# Autodesk Inventor assembly: left arm
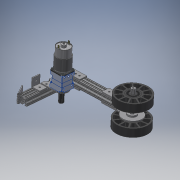
[picture p0: Inventor's stored thumbnail of the model, 180x180]
Saved by Autodesk Inventor 2018 (Build 220112000, 112)
## iProperties
Created: 2019-01-25
Part Number: left arm
Document SubType Name: Assembly
Designer: s-2513225
Author: s-2513225
## Documents named in this file (12)
- E:\Robotics\Ball Intake ver 2\left arm.iam
- E:\Robotics\Ball Intake ver 2\1010 6in.ipt
- E:\Robotics\Ball Intake ver 2\1010 7in.ipt
- E:\Robotics\Ball Intake ver 2\motor connector.ipt
- E:\Robotics\Ball Intake ver 2\VersaPlanetary_v1_Single_Stage_10_1_with_775_Series.ipt
- E:\Robotics\Ball Intake ver 2\wheel tip.ipt
- E:\Robotics\Ball Intake ver 2\0_500_ID_x_1_125_OD_x_0_313_WD_Flanged_Bearing_217-2731.ipt
- E:\Robotics\Ball Intake ver 2\1_2_Hex_x_0_201_ID_ThunderHex_Stock_18_217-4002.ipt
- E:\Robotics\Ball Intake ver 2\am-3480 4IN 500Hex Bore Compliant Wheel.ipt
- E:\Robotics\Ball Intake ver 2\hinge.ipt
- E:\Robotics\Ball Intake ver 2\8020 connector.ipt
- E:\Robotics\Ball Intake ver 2\spring connector.ipt
## Components (17 placed, 11 different names)
1. 1010 6in:1 — Mate:4, Flush:12, Mate:11, Flush:13, Flush:14, Mate:18, Flush:15, Flush:17, Flush:18, Mate:21, Flush:20, Mate:22, Flush:22
2. 1010 7in:1 — Mate:2, Flush:3, Flush:4, Mate:3, Flush:5, Flush:6, Mate:11, Flush:13, Flush:14, Mate:20, Flush:19, Flush:21
3. motor connector:1 — Mate:4, Mate:5, Flush:9, Flush:12
4. VersaPlanetary_v1_Single_Stage_10_1_with_775_Series:1 — Mate:12, Mate:13
5. wheel tip:1 — Mate:2, Flush:3, Flush:4, Flush:7, Mate:7, Flush:11
6. wheel tip:2 — Mate:3, Flush:5, Flush:6, Flush:7, Mate:6, Flush:10
7. 0_500_ID_x_1_125_OD_x_0_313_WD_Flanged_Bearing_217-2731:1 — Mate:5, Flush:9, Mate:12, Mate:13
8. 0_500_ID_x_1_125_OD_x_0_313_WD_Flanged_Bearing_217-2731:2 — Mate:7, Flush:11, Mate:10
9. 0_500_ID_x_1_125_OD_x_0_313_WD_Flanged_Bearing_217-2731:3 — Mate:6, Flush:10
10. 1_2_Hex_x_0_201_ID_ThunderHex_Stock_18_217-4002:1 — Mate:10, Mate:14, Mate:15, Mate:16, Mate:17
11. am-3480 4IN 500Hex Bore Compliant Wheel:1 — Mate:14, Mate:15
12. am-3480 4IN 500Hex Bore Compliant Wheel:2 — Mate:16, Mate:17
13. hinge:1 — Mate:18, Flush:15, Mate:19, Flush:16, Flush:17
14. hinge:2 — Mate:19, Flush:16
15. 8020 connector:1 — Mate:20, Flush:18, Flush:19
16. 8020 connector:2 — Mate:21, Flush:20, Flush:21
17. spring connector:1 — Mate:22, Flush:22
## Relationships (38: Mate 19, Flush 19)
- Mate:2: 1010 7in:1 ↔ wheel tip:1
- Flush:3: 1010 7in:1 ↔ wheel tip:1
- Flush:4: 1010 7in:1 ↔ wheel tip:1
- Mate:3: 1010 7in:1 ↔ wheel tip:2
- Flush:5: 1010 7in:1 ↔ wheel tip:2
- Flush:6: 1010 7in:1 ↔ wheel tip:2
- Flush:7: wheel tip:1 ↔ wheel tip:2
- Mate:4: 1010 6in:1 ↔ motor connector:1
- Mate:5: motor connector:1 ↔ 0_500_ID_x_1_125_OD_x_0_313_WD_Flanged_Bearing_217-2731:1
- Flush:9: motor connector:1 ↔ 0_500_ID_x_1_125_OD_x_0_313_WD_Flanged_Bearing_217-2731:1
- Mate:6: wheel tip:2 ↔ 0_500_ID_x_1_125_OD_x_0_313_WD_Flanged_Bearing_217-2731:3
- Flush:10: wheel tip:2 ↔ 0_500_ID_x_1_125_OD_x_0_313_WD_Flanged_Bearing_217-2731:3
- Mate:7: wheel tip:1 ↔ 0_500_ID_x_1_125_OD_x_0_313_WD_Flanged_Bearing_217-2731:2
- Flush:11: wheel tip:1 ↔ 0_500_ID_x_1_125_OD_x_0_313_WD_Flanged_Bearing_217-2731:2
- Mate:10: 0_500_ID_x_1_125_OD_x_0_313_WD_Flanged_Bearing_217-2731:2 ↔ 1_2_Hex_x_0_201_ID_ThunderHex_Stock_18_217-4002:1
- Flush:12: 1010 6in:1 ↔ motor connector:1
- Mate:11: 1010 6in:1 ↔ 1010 7in:1
- Flush:13: 1010 6in:1 ↔ 1010 7in:1
- Flush:14: 1010 6in:1 ↔ 1010 7in:1
- Mate:12: VersaPlanetary_v1_Single_Stage_10_1_with_775_Series:1 ↔ 0_500_ID_x_1_125_OD_x_0_313_WD_Flanged_Bearing_217-2731:1
- Mate:13: VersaPlanetary_v1_Single_Stage_10_1_with_775_Series:1 ↔ 0_500_ID_x_1_125_OD_x_0_313_WD_Flanged_Bearing_217-2731:1
- Mate:14: 1_2_Hex_x_0_201_ID_ThunderHex_Stock_18_217-4002:1 ↔ am-3480 4IN 500Hex Bore Compliant Wheel:1
- Mate:15: 1_2_Hex_x_0_201_ID_ThunderHex_Stock_18_217-4002:1 ↔ am-3480 4IN 500Hex Bore Compliant Wheel:1
- Mate:16: 1_2_Hex_x_0_201_ID_ThunderHex_Stock_18_217-4002:1 ↔ am-3480 4IN 500Hex Bore Compliant Wheel:2
- Mate:17: 1_2_Hex_x_0_201_ID_ThunderHex_Stock_18_217-4002:1 ↔ am-3480 4IN 500Hex Bore Compliant Wheel:2
- Mate:18: 1010 6in:1 ↔ hinge:1
- Flush:15: 1010 6in:1 ↔ hinge:1
- Mate:19: hinge:1 ↔ hinge:2
- Flush:16: hinge:1 ↔ hinge:2
- Flush:17: 1010 6in:1 ↔ hinge:1
- Mate:20: 1010 7in:1 ↔ 8020 connector:1
- Flush:18: 1010 6in:1 ↔ 8020 connector:1
- Flush:19: 1010 7in:1 ↔ 8020 connector:1
- Mate:21: 1010 6in:1 ↔ 8020 connector:2
- Flush:20: 1010 6in:1 ↔ 8020 connector:2
- Flush:21: 1010 7in:1 ↔ 8020 connector:2
- Mate:22: 1010 6in:1 ↔ spring connector:1
- Flush:22: 1010 6in:1 ↔ spring connector:1
